# Autodesk Inventor assembly: wheel kenda turf tire
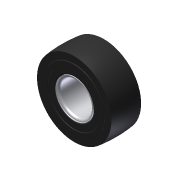
[picture p0: Inventor's stored thumbnail of the model, 180x180]
Saved by Autodesk Inventor 2012 (Build 160160000, 160)
## iProperties
Created: 2011-11-26
Part Number: wheel kenda turf tire
Document SubType Name: Assembly
Designer: Antonella
Author: Antonella
## Documents named in this file (4)
- C:\Users\Antonella\Documents\GCC Robotics 2012 - Mechanical\Robot 2.0\Drive Train\Turf Tire\wheel kenda turf tire.iam
- C:\Users\Antonella\Documents\GCC Robotics 2012 - Mechanical\Robot 2.0\Drive Train\Turf Tire\rim_8 in x 6.3 in.ipt
- C:\Users\Antonella\Documents\GCC Robotics 2012 - Mechanical\Robot 2.0\Drive Train\Turf Tire\tire 16.2 od.ipt
- C:\Users\Antonella\Documents\GCC Robotics 2012 - Mechanical\Robot 2.0\Drive Train\Turf Tire\wheel hub.ipt
## Components (3 placed, 3 different names)
1. rim_8 in x 6.3 in:1 — Mate:1, Mate:2, Mate:4, Mate:5
2. tire 16.2 od:1 — Mate:1, Mate:2
3. wheel hub:1 — Mate:4, Mate:5
## Relationships (4: Mate 4)
- Mate:1: rim_8 in x 6.3 in:1 ↔ tire 16.2 od:1
- Mate:2: rim_8 in x 6.3 in:1 ↔ tire 16.2 od:1
- Mate:4: rim_8 in x 6.3 in:1 ↔ wheel hub:1
- Mate:5: rim_8 in x 6.3 in:1 ↔ wheel hub:1
